# Autodesk Inventor assembly: SS-01GL13-E
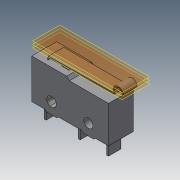
[picture p0: Inventor's stored thumbnail of the model, 180x180]
Saved by Autodesk Inventor 2018.3 (Build 223284000, 284)
## iProperties
Created: 2016-03-28
Vendor: HHMI: JRC - ID&F
Document SubType Name: Assembly
Designer: ARNOLDJ
RuleStatus: InUse
AfterDocSave0: file://Part Number Cleaner
DESIGN DEPARTMENT: HHMI: JRC - ID&F
ALTERED ITEM PART NUMBER: N/A
ALTERED ITEM VENDOR: N/A
ALTERED ITEM DESCRIPTION: N/A
Author: ARNOLDJ
Revision Number: 0
## Documents named in this file (3)
- C:\_WORKSPACE\DATA\COMMON\OMRON\SS-01GL13-E.iam
- C:\_WORKSPACE\DATA\COMMON\OMRON\SS_01GL13_E.ipt
- C:\_WORKSPACE\DATA\COMMON\OMRON\SS_01GL13_E_lever.ipt
## Components (2 placed, 2 different names)
1. SS_01GL13_E:1 — Flush:1, Mate:1, Flush:2, Mate:2
2. SS_01GL13_E_lever:1 — Flush:1, Mate:1, Tangent:1
## Relationships (8: Flush 4, Mate 2, Tangent 1, Angle 1)
- Flush:1: SS_01GL13_E:1 ↔ SS_01GL13_E_lever:1
- Mate:1: SS_01GL13_E:1 ↔ SS_01GL13_E_lever:1
- Flush:2 (10.7 mm): SS_01GL13_E:1
- Tangent:1: SS_01GL13_E_lever:1
- Flush:3 (0.8 mm)
- Flush:4 (-0.8 mm)
- Mate:2: SS_01GL13_E:1
- Angle:1 (0 deg)
